# Autodesk Inventor assembly: Slides Bearings
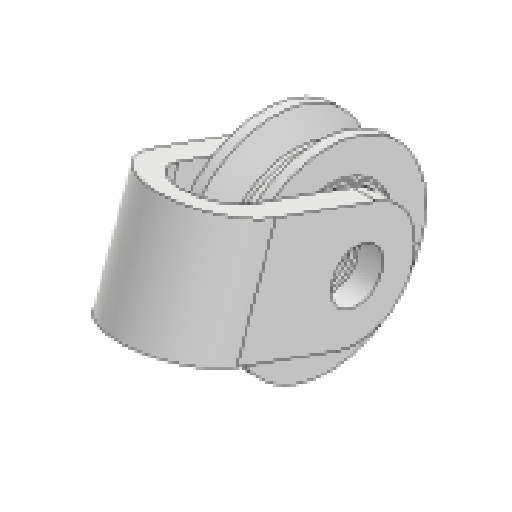
[picture p0: Inventor's stored thumbnail of the model, 512x512]
Saved by Autodesk Inventor 2023 (Build 270158000, 158)
## iProperties
Created: 2022-10-19
Part Number: Slides Bearings
Document SubType Name: Assembly
Designer: deli
Author: deli
## Documents named in this file (3)
- C:\Users\deli\OneDrive - Eastside Preparatory School\FTC\8103-power-play\CAD\Slides Bearings.iam
- C:\Users\deli\OneDrive - Eastside Preparatory School\FTC\8103-power-play\CAD\FTC-parts\LongRobotics\3x12x4mm-bearing.ipt
- C:\Users\deli\OneDrive - Eastside Preparatory School\FTC\8103-power-play\CAD\Bearing covers.ipt
## Components (2 placed, 2 different names)
1. 3x12x4mm-bearing:1 — Mate:1, Mate:2
2. Bearing covers:1 — Mate:1, Mate:2
## Relationships (2: Mate 2)
- Mate:1: 3x12x4mm-bearing:1 ↔ Bearing covers:1
- Mate:2 (0.25 mm): 3x12x4mm-bearing:1 ↔ Bearing covers:1
